# Autodesk Inventor assembly: Z Idler A
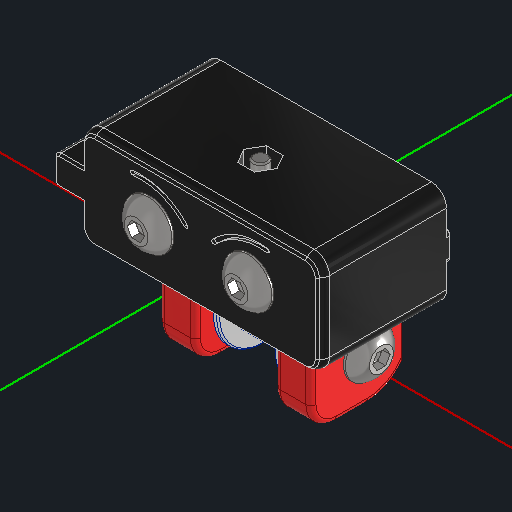
[picture p0: Inventor's stored thumbnail of the model, 512x512]
Saved by Autodesk Inventor 2022.2 (Build 262287010, 287A)
## iProperties
Created: 2022-03-12
Part Number: Z Idler A
Document SubType Name: Assembly
Designer: sleib
Author: sleib
## Documents named in this file (7)
- C:\Users\sleib\Projekte\Voron-2\CAD\Inventor\Z Idler [A].iam
- C:\Users\sleib\Projekte\Voron-2\CAD\Inventor\Z Idler-Body [A].ipt
- C:\Users\sleib\Projekte\Voron-2\CAD\Inventor\M3 Hexnut.ipt
- C:\Users\sleib\Projekte\Voron-2\CAD\Inventor\Z Idler-Tensioner (9mm).ipt
- C:\Users\sleib\Projekte\Voron-2\CAD\Inventor\M3x16 SHCS.ipt
- C:\Users\sleib\Projekte\Voron-2\CAD\Inventor\M5x30 BHCS.ipt
- C:\Users\sleib\Projekte\Voron-2\CAD\Inventor\GT2 20T Idler (9mm).ipt
## Components (8 placed, 6 different names)
1. Z Idler-Body [A]:1 — Passend:1, Fluchtend:1, Passend:2, Passend:3, Passend:4, Winkel:1, Winkel:2, Passend:13, Passend:14, Passend:15, Passend:16, Passend:17
2. Z Idler-Tensioner (9mm):1 — Passend:6, Passend:7, Winkel:2, Passend:9, Passend:10, Passend:12, Passend:17
3. GT2 20T Idler (9mm):1 — Passend:11, Passend:12
4. M3 Hexnut:1 — Passend:3, Passend:4, Winkel:1, Passend:8
5. M3x16 SHCS:1 — Passend:6, Passend:7, Passend:8
6. M5x30 BHCS:1 — Passend:9, Passend:10, Passend:11
7. M5x30 BHCS:2 — Passend:13, Passend:15
8. M5x30 BHCS:3 — Passend:14, Passend:16
## Relationships (19: Mate 16, Angle 2, Flush 1)
- Passend:1 [Mate]: Z Idler-Body [A]:1
- Fluchtend:1 [Flush]: Z Idler-Body [A]:1
- Passend:2 [Mate]: Z Idler-Body [A]:1
- Passend:3 [Mate]: Z Idler-Body [A]:1 ↔ M3 Hexnut:1
- Passend:4 [Mate]: Z Idler-Body [A]:1 ↔ M3 Hexnut:1
- Winkel:1 [Angle] (0 deg): Z Idler-Body [A]:1 ↔ M3 Hexnut:1
- Passend:6 [Mate]: Z Idler-Tensioner (9mm):1 ↔ M3x16 SHCS:1
- Passend:7 [Mate]: Z Idler-Tensioner (9mm):1 ↔ M3x16 SHCS:1
- Passend:8 [Mate]: M3 Hexnut:1 ↔ M3x16 SHCS:1
- Winkel:2 [Angle] (0 deg): Z Idler-Body [A]:1 ↔ Z Idler-Tensioner (9mm):1
- Passend:9 [Mate]: Z Idler-Tensioner (9mm):1 ↔ M5x30 BHCS:1
- Passend:10 [Mate]: Z Idler-Tensioner (9mm):1 ↔ M5x30 BHCS:1
- Passend:11 [Mate]: GT2 20T Idler (9mm):1 ↔ M5x30 BHCS:1
- Passend:12 [Mate] (1.4 mm): Z Idler-Tensioner (9mm):1 ↔ GT2 20T Idler (9mm):1
- Passend:13 [Mate]: Z Idler-Body [A]:1 ↔ M5x30 BHCS:2
- Passend:14 [Mate]: Z Idler-Body [A]:1 ↔ M5x30 BHCS:3
- Passend:15 [Mate]: Z Idler-Body [A]:1 ↔ M5x30 BHCS:2
- Passend:16 [Mate]: Z Idler-Body [A]:1 ↔ M5x30 BHCS:3
- Passend:17 [Mate]: Z Idler-Body [A]:1 ↔ Z Idler-Tensioner (9mm):1
